# Autodesk Inventor assembly: robot2
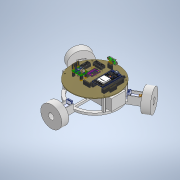
[picture p0: Inventor's stored thumbnail of the model, 180x180]
Saved by Autodesk Inventor 2020 (Build 240168000, 168)
## iProperties
Created: 2020-03-23
Part Number: robot2
Document SubType Name: Assembly
Designer: Tarsoly
Author: Tarsoly
## Documents named in this file (22)
- D:\Users\Tarsoly\Dokumentumok\BME\8. Félév\Önlab\3d\robot2.iam
- D:\Users\Tarsoly\Dokumentumok\BME\8. Félév\Önlab\3d\bottom2.ipt
- D:\Users\Tarsoly\Dokumentumok\BME\8. Félév\Önlab\3d\omniwheel.ipt
- D:\Users\Tarsoly\Dokumentumok\BME\8. Félév\Önlab\3d\DC_GE_Motor\DC_GE_RED_Motor.iam
- D:\Users\Tarsoly\Dokumentumok\BME\8. Félév\Önlab\3d\akksi.ipt
- D:\Users\Tarsoly\Dokumentumok\BME\8. Félév\Önlab\3d\PCB\main_board.iam
- D:\Users\Tarsoly\Dokumentumok\BME\8. Félév\Önlab\3d\tavtarto_30mm.ipt
- D:\Users\Tarsoly\Dokumentumok\BME\8. Félév\Önlab\3d\pins\socket\10x1\FH01-10SS.iam
- D:\Users\Tarsoly\Dokumentumok\BME\8. Félév\Önlab\3d\pins\socket\9x1\FH01-09SS.iam
- D:\Users\Tarsoly\Dokumentumok\BME\8. Félév\Önlab\3d\ESP32\ESP32S Dev Board 0.9inch width ASSY_TOP.iam
- D:\Users\Tarsoly\Dokumentumok\BME\8. Félév\Önlab\3d\PCB_v2\main_board.iam
- D:\Users\Tarsoly\Dokumentumok\BME\8. Félév\Önlab\3d\pins\socket\6x1\FH01-06SS.iam
- D:\Users\Tarsoly\Dokumentumok\BME\8. Félév\Önlab\3d\pins\dip_socket\IC_Sockel_16P.ipt
- D:\Users\Tarsoly\Dokumentumok\BME\8. Félév\Önlab\3d\L293D\L293D v1.iam
- D:\Users\Tarsoly\Dokumentumok\BME\8. Félév\Önlab\3d\pins\socket\4x1\FH01-04SS.iam
- D:\Users\Tarsoly\Dokumentumok\BME\8. Félév\Önlab\3d\pins\socket\3x1\FH01-03SS.iam
- D:\Users\Tarsoly\Dokumentumok\BME\8. Félév\Önlab\3d\pins\socket\2x1\FH01-02SS.iam
- D:\Users\Tarsoly\Dokumentumok\BME\8. Félév\Önlab\3d\pins\header\Pin Header 1x2 TH Pitch 2.54mm.ipt
- D:\Users\Tarsoly\Dokumentumok\BME\8. Félév\Önlab\3d\pins\header\Pin Header 1x4 TH Angle Pitch 2.54mm.ipt
- D:\Users\Tarsoly\Dokumentumok\BME\8. Félév\Önlab\3d\MPU2950\GY-91.iam
- D:\Users\Tarsoly\Dokumentumok\BME\8. Félév\Önlab\3d\VL5310X\vl53l0x.ipt
- D:\Users\Tarsoly\Dokumentumok\BME\8. Félév\Önlab\3d\DSN-1504\DC-DC 4.5-28V to 0.8-20V Output 3A MP1584EN Step Down Buck Converter_TOP.iam
## Components (45 placed, 20 different names)
1. bottom2:1 — Mate:1, Flush:3, Flush:4, Mate:14, Mate:15, Mate:16, Mate:17, Mate:18, Mate:19, Mate:20, Mate:21, Mate:22, Mate:23, Mate:24, Mate:25, Mate:29, Mate:30, Mate:31, Mate:32, Mate:33, Mate:34, Mate:35, Mate:36, Mate:37, Mate:38
2. omniwheel:1 — Mate:14, Mate:26
3. omniwheel:2 — Mate:16, Mate:27
4. omniwheel:3 — Mate:15, Mate:28
5. DC_GE_RED_Motor:1 [sub-assembly] — Mate:19, Mate:22, Mate:23, Mate:26
6. DC_GE_RED_Motor:2 [sub-assembly] — Mate:17, Mate:20, Mate:24, Mate:28
7. DC_GE_RED_Motor:3 [sub-assembly] — Mate:18, Mate:21, Mate:25, Mate:27
8. akksi:1 — Mate:29, Mate:30
9. main_board:1 [sub-assembly] — Mate:39, Mate:40, Angle:1, Mate:41, Mate:44, Mate:47, Mate:50
10. tavtarto_30mm:1 — Mate:31, Mate:32, Mate:39
11. tavtarto_30mm:2 — Mate:33, Mate:37, Mate:40, Mate:57
12. tavtarto_30mm:3 — Mate:34, Mate:38
13. tavtarto_30mm:4 — Mate:35, Mate:36, Mate:56
14. FH01-10SS:1 [sub-assembly] — Mate:41, Mate:60, Mate:61
15. FH01-10SS:2 [sub-assembly] — Mate:44, Mate:64, Mate:65
16. FH01-09SS:1 [sub-assembly] — Mate:47, Mate:55, Mate:58, Mate:59
17. FH01-09SS:2 [sub-assembly] — Mate:50, Flush:5, Flush:6, Mate:62, Mate:63
18. ESP32S Dev Board 0.9inch width ASSY_TOP:1 [sub-assembly] — Mate:55, Flush:5, Flush:6
19. main_board:2 [sub-assembly] — Mate:56, Mate:57, Mate:58, Mate:59, Mate:60, Mate:61, Angle:2, Mate:62, Mate:63, Mate:64, Mate:65, Mate:66, Mate:67, Mate:68, Mate:69, Mate:70, Mate:71, Mate:72, Mate:73, Mate:74, Mate:75, Mate:76, Mate:77, Mate:78, Mate:79, Mate:80, Mate:81, Mate:82, Mate:83, Mate:84, Mate:85, Mate:86, Mate:87, Mate:88, Mate:89, Mate:90, Mate:91, Mate:92, Mate:99, Mate:100, Mate:101, Mate:102, Mate:103, Mate:104, Mate:105, Mate:106, Mate:107, Mate:108, Mate:109, Mate:110, Mate:111, Mate:112, Mate:113, Mate:114, Mate:115, Mate:116, Mate:117, Mate:125
20. FH01-10SS:3 [sub-assembly] — Mate:66, Mate:67, Mate:68
21. FH01-09SS:3 [sub-assembly] — Mate:69, Mate:70, Mate:71
22. FH01-10SS:4 [sub-assembly] — Mate:75, Mate:76, Mate:77
23. FH01-09SS:4 [sub-assembly] — Mate:72, Mate:73, Mate:74
24. FH01-06SS:1 [sub-assembly] — Mate:78, Mate:79, Mate:80
25. FH01-06SS:2 [sub-assembly] — Mate:81, Mate:82, Mate:83
26. FH01-06SS:3 [sub-assembly] — Mate:84, Mate:85, Mate:86
27. IC_Sockel_16P:1 — Mate:87, Mate:88, Mate:89, Mate:93, Mate:94, Mate:95
28. IC_Sockel_16P:2 — Mate:90, Mate:91, Mate:92, Mate:96, Mate:97, Mate:98
29. L293D v1:1 [sub-assembly] — Mate:93, Mate:94, Mate:95
30. L293D v1:2 [sub-assembly] — Mate:96, Mate:97, Mate:98
31. FH01-04SS:1 [sub-assembly] — Mate:99, Mate:100, Mate:101, Mate:120, Mate:121, Angle:6
32. FH01-04SS:2 [sub-assembly] — Mate:102, Mate:103, Mate:104, Mate:122, Flush:7, Flush:8
33. FH01-03SS:1 [sub-assembly] — Mate:105, Mate:106, Mate:107
34. FH01-02SS:1 [sub-assembly] — Mate:109, Mate:110, Mate:111
35. FH01-02SS:2 [sub-assembly] — Mate:108, Mate:112, Mate:113, Mate:134, Mate:135, Angle:7
36. Pin Header 1x2 TH Pitch 2.54mm:1 — Mate:115, Mate:117, Angle:4
37. Pin Header 1x2 TH Pitch 2.54mm:2 — Mate:114, Mate:116, Angle:3
38. Pin Header 1x4 TH Angle Pitch 2.54mm:1 — Mate:120, Mate:121, Angle:6, Mate:123, Mate:124
39. FH01-02SS:3 [sub-assembly] — Mate:127, Mate:129, Flush:9
40. FH01-02SS:4 [sub-assembly] — Mate:126, Mate:128, Flush:10
41. GY-91:1 [sub-assembly] — Mate:122, Flush:7, Flush:8
42. vl53l0x:1 — Mate:123, Mate:124, Mate:125
43. DC-DC 4.5-28V to 0.8-20V Output 3A MP1584EN Step Down Buck Converter_TOP:1 [sub-assembly] — Mate:126, Mate:127, Mate:128, Mate:129, Flush:9, Flush:10, Mate:130, Mate:131, Mate:132, Mate:133, Flush:11, Flush:12
44. Pin Header 1x2 TH Pitch 2.54mm:3 — Mate:130, Mate:133, Flush:11, Mate:135
45. Pin Header 1x2 TH Pitch 2.54mm:4 — Mate:131, Mate:132, Flush:12, Mate:134, Angle:7
## Relationships (127: Mate 111, Flush 10, Angle 6)
- Mate:1: bottom2:1
- Flush:3 (-2 mm): bottom2:1
- Flush:4 (-2 mm): bottom2:1
- Mate:14 (1 mm): bottom2:1 ↔ omniwheel:1
- Mate:15 (1 mm): bottom2:1 ↔ omniwheel:3
- Mate:16 (1 mm): bottom2:1 ↔ omniwheel:2
- Mate:17: bottom2:1 ↔ DC_GE_RED_Motor:2
- Mate:18: bottom2:1 ↔ DC_GE_RED_Motor:3
- Mate:19: bottom2:1 ↔ DC_GE_RED_Motor:1
- Mate:20: bottom2:1 ↔ DC_GE_RED_Motor:2
- Mate:21: bottom2:1 ↔ DC_GE_RED_Motor:3
- Mate:22: bottom2:1 ↔ DC_GE_RED_Motor:1
- Mate:23 (1 mm): bottom2:1 ↔ DC_GE_RED_Motor:1
- Mate:24 (1 mm): bottom2:1 ↔ DC_GE_RED_Motor:2
- Mate:25 (1 mm): bottom2:1 ↔ DC_GE_RED_Motor:3
- Mate:26: omniwheel:1 ↔ DC_GE_RED_Motor:1
- Mate:27: omniwheel:2 ↔ DC_GE_RED_Motor:3
- Mate:28: omniwheel:3 ↔ DC_GE_RED_Motor:2
- Mate:29: bottom2:1 ↔ akksi:1
- Mate:30 (0.5 mm): bottom2:1 ↔ akksi:1
- Mate:31: bottom2:1 ↔ tavtarto_30mm:1
- Mate:32: bottom2:1 ↔ tavtarto_30mm:1
- Mate:33: bottom2:1 ↔ tavtarto_30mm:2
- Mate:34: bottom2:1 ↔ tavtarto_30mm:3
- Mate:35: bottom2:1 ↔ tavtarto_30mm:4
- Mate:36: bottom2:1 ↔ tavtarto_30mm:4
- Mate:37: bottom2:1 ↔ tavtarto_30mm:2
- Mate:38: bottom2:1 ↔ tavtarto_30mm:3
- Mate:39: main_board:1 ↔ tavtarto_30mm:1
- Mate:40: main_board:1 ↔ tavtarto_30mm:2
- Angle:1 (180 deg): main_board:1
- Mate:41: main_board:1 ↔ FH01-10SS:1
- Mate:44: main_board:1 ↔ FH01-10SS:2
- Mate:47: main_board:1 ↔ FH01-09SS:1
- Mate:50: main_board:1 ↔ FH01-09SS:2
- Mate:55: FH01-09SS:1 ↔ ESP32S Dev Board 0.9inch width ASSY_TOP:1
- Flush:5: FH01-09SS:2 ↔ ESP32S Dev Board 0.9inch width ASSY_TOP:1
- Flush:6: FH01-09SS:2 ↔ ESP32S Dev Board 0.9inch width ASSY_TOP:1
- Mate:56: tavtarto_30mm:4 ↔ main_board:2
- Mate:57: tavtarto_30mm:2 ↔ main_board:2
- Mate:58: FH01-09SS:1 ↔ main_board:2
- Mate:59: FH01-09SS:1 ↔ main_board:2
- Mate:60: FH01-10SS:1 ↔ main_board:2
- Mate:61: FH01-10SS:1 ↔ main_board:2
- Angle:2 (180 deg): main_board:2
- Mate:62: FH01-09SS:2 ↔ main_board:2
- Mate:63: FH01-09SS:2 ↔ main_board:2
- Mate:64: FH01-10SS:2 ↔ main_board:2
- Mate:65: FH01-10SS:2 ↔ main_board:2
- Mate:66: main_board:2 ↔ FH01-10SS:3
- Mate:67: main_board:2 ↔ FH01-10SS:3
- Mate:68: main_board:2 ↔ FH01-10SS:3
- Mate:69: main_board:2 ↔ FH01-09SS:3
- Mate:70: main_board:2 ↔ FH01-09SS:3
- Mate:71: main_board:2 ↔ FH01-09SS:3
- Mate:72: main_board:2 ↔ FH01-09SS:4
- Mate:73: main_board:2 ↔ FH01-09SS:4
- Mate:74: main_board:2 ↔ FH01-09SS:4
- Mate:75: main_board:2 ↔ FH01-10SS:4
- Mate:76: main_board:2 ↔ FH01-10SS:4
- Mate:77: main_board:2 ↔ FH01-10SS:4
- Mate:78: main_board:2 ↔ FH01-06SS:1
- Mate:79: main_board:2 ↔ FH01-06SS:1
- Mate:80: main_board:2 ↔ FH01-06SS:1
- Mate:81: main_board:2 ↔ FH01-06SS:2
- Mate:82: main_board:2 ↔ FH01-06SS:2
- Mate:83: main_board:2 ↔ FH01-06SS:2
- Mate:84: main_board:2 ↔ FH01-06SS:3
- Mate:85: main_board:2 ↔ FH01-06SS:3
- Mate:86: main_board:2 ↔ FH01-06SS:3
- Mate:87: main_board:2 ↔ IC_Sockel_16P:1
- Mate:88: main_board:2 ↔ IC_Sockel_16P:1
- Mate:89: main_board:2 ↔ IC_Sockel_16P:1
- Mate:90: main_board:2 ↔ IC_Sockel_16P:2
- Mate:91: main_board:2 ↔ IC_Sockel_16P:2
- Mate:92: main_board:2 ↔ IC_Sockel_16P:2
- Mate:93: IC_Sockel_16P:1 ↔ L293D v1:1
- Mate:94: IC_Sockel_16P:1 ↔ L293D v1:1
- Mate:95 (-1.522 mm): IC_Sockel_16P:1 ↔ L293D v1:1
- Mate:96: IC_Sockel_16P:2 ↔ L293D v1:2
- Mate:97: IC_Sockel_16P:2 ↔ L293D v1:2
- Mate:98 (-1.518 mm): IC_Sockel_16P:2 ↔ L293D v1:2
- Mate:99: main_board:2 ↔ FH01-04SS:1
- Mate:100: main_board:2 ↔ FH01-04SS:1
- Mate:101: main_board:2 ↔ FH01-04SS:1
- Mate:102: main_board:2 ↔ FH01-04SS:2
- Mate:103: main_board:2 ↔ FH01-04SS:2
- Mate:104: main_board:2 ↔ FH01-04SS:2
- Mate:105: main_board:2 ↔ FH01-03SS:1
- Mate:106: main_board:2 ↔ FH01-03SS:1
- Mate:107: main_board:2 ↔ FH01-03SS:1
- Mate:108: main_board:2 ↔ FH01-02SS:2
- Mate:109: main_board:2 ↔ FH01-02SS:1
- Mate:110: main_board:2 ↔ FH01-02SS:1
- Mate:111: main_board:2 ↔ FH01-02SS:1
- Mate:112: main_board:2 ↔ FH01-02SS:2
- Mate:113: main_board:2 ↔ FH01-02SS:2
- Mate:114: main_board:2 ↔ Pin Header 1x2 TH Pitch 2.54mm:2
- Mate:115: main_board:2 ↔ Pin Header 1x2 TH Pitch 2.54mm:1
- Mate:116: main_board:2 ↔ Pin Header 1x2 TH Pitch 2.54mm:2
- Angle:3 (180 deg): Pin Header 1x2 TH Pitch 2.54mm:2
- Mate:117: main_board:2 ↔ Pin Header 1x2 TH Pitch 2.54mm:1
- Angle:4 (0 deg): Pin Header 1x2 TH Pitch 2.54mm:1
- Mate:120: FH01-04SS:1 ↔ Pin Header 1x4 TH Angle Pitch 2.54mm:1
- Mate:121: FH01-04SS:1 ↔ Pin Header 1x4 TH Angle Pitch 2.54mm:1
- Angle:6 (180 deg): FH01-04SS:1 ↔ Pin Header 1x4 TH Angle Pitch 2.54mm:1
- Mate:122: FH01-04SS:2 ↔ GY-91:1
- Flush:7: FH01-04SS:2 ↔ GY-91:1
- Flush:8: FH01-04SS:2 ↔ GY-91:1
- Mate:123: Pin Header 1x4 TH Angle Pitch 2.54mm:1 ↔ vl53l0x:1
- Mate:124: Pin Header 1x4 TH Angle Pitch 2.54mm:1 ↔ vl53l0x:1
- Mate:125 (11.12 mm): main_board:2 ↔ vl53l0x:1
- Mate:126: FH01-02SS:4 ↔ DC-DC 4.5-28V to 0.8-20V Output 3A MP1584EN Step Down Buck Converter_TOP:1
- Mate:127: FH01-02SS:3 ↔ DC-DC 4.5-28V to 0.8-20V Output 3A MP1584EN Step Down Buck Converter_TOP:1
- Mate:128: FH01-02SS:4 ↔ DC-DC 4.5-28V to 0.8-20V Output 3A MP1584EN Step Down Buck Converter_TOP:1
- Mate:129: FH01-02SS:3 ↔ DC-DC 4.5-28V to 0.8-20V Output 3A MP1584EN Step Down Buck Converter_TOP:1
- Flush:9 (0.55 mm): FH01-02SS:3 ↔ DC-DC 4.5-28V to 0.8-20V Output 3A MP1584EN Step Down Buck Converter_TOP:1
- Flush:10 (0.55 mm): FH01-02SS:4 ↔ DC-DC 4.5-28V to 0.8-20V Output 3A MP1584EN Step Down Buck Converter_TOP:1
- Mate:130: DC-DC 4.5-28V to 0.8-20V Output 3A MP1584EN Step Down Buck Converter_TOP:1 ↔ Pin Header 1x2 TH Pitch 2.54mm:3
- Mate:131: DC-DC 4.5-28V to 0.8-20V Output 3A MP1584EN Step Down Buck Converter_TOP:1 ↔ Pin Header 1x2 TH Pitch 2.54mm:4
- Mate:132: DC-DC 4.5-28V to 0.8-20V Output 3A MP1584EN Step Down Buck Converter_TOP:1 ↔ Pin Header 1x2 TH Pitch 2.54mm:4
- Mate:133: DC-DC 4.5-28V to 0.8-20V Output 3A MP1584EN Step Down Buck Converter_TOP:1 ↔ Pin Header 1x2 TH Pitch 2.54mm:3
- Flush:11 (0.53 mm): DC-DC 4.5-28V to 0.8-20V Output 3A MP1584EN Step Down Buck Converter_TOP:1 ↔ Pin Header 1x2 TH Pitch 2.54mm:3
- Flush:12 (0.53 mm): DC-DC 4.5-28V to 0.8-20V Output 3A MP1584EN Step Down Buck Converter_TOP:1 ↔ Pin Header 1x2 TH Pitch 2.54mm:4
- Mate:134: FH01-02SS:2 ↔ Pin Header 1x2 TH Pitch 2.54mm:4
- Mate:135: FH01-02SS:2 ↔ Pin Header 1x2 TH Pitch 2.54mm:3
- Angle:7 (180 deg): FH01-02SS:2 ↔ Pin Header 1x2 TH Pitch 2.54mm:4
